# Autodesk Inventor assembly: 27t track drive sprocket
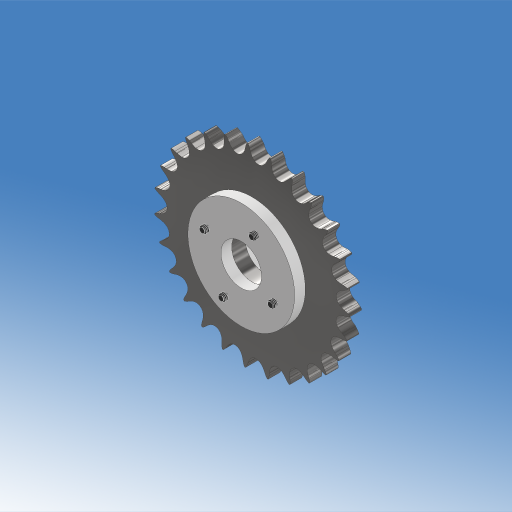
[picture p0: Inventor's stored thumbnail of the model, 512x512]
Saved by Autodesk Inventor 2024 (Build 280153000, 153)
## iProperties
Created: 2023-01-21
Part Number: 27t track drive sprocket
Document SubType Name: Assembly
Designer: AdminForWorker
Title: 27t track drive sprocket v25
Author: AdminForWorker
## Documents named in this file (5)
- C:\Users\seene\OneDrive\SBRT\Robocup Rescue\Drive\v1\TANK flipper\27t track drive sprocket v25.iam
- C:\Users\seene\OneDrive\SBRT\Robocup Rescue\Drive\v1\TANK flipper\91259A166_Alloy Steel Shoulder Screw v2.ipt
- C:\Users\seene\OneDrive\SBRT\Robocup Rescue\Drive\v1\TANK flipper\sprocket.ipt
- C:\Users\seene\OneDrive\SBRT\Robocup Rescue\Drive\v1\flipper dxf\drive sprocket flange.ipt
- C:\Users\seene\OneDrive\SBRT\Robocup Rescue\Drive\v1\flipper dxf\drive sprocket flange socket.ipt
## Components (7 placed, 4 different names)
1. 91259A166_Alloy Steel Shoulder Screw v2:5 — Rigid:4
2. 91259A166_Alloy Steel Shoulder Screw v2:6 — Rigid:3
3. 91259A166_Alloy Steel Shoulder Screw v2:7 — Rigid:2
4. 91259A166_Alloy Steel Shoulder Screw v2:8 — Rigid:1
5. sprocket:1 — Mate:1, Mate:2, Mate:3, Mate:4, Rigid:1, Rigid:2, Rigid:3, Rigid:4
6. drive sprocket flange:1 — Mate:3, Mate:4
7. drive sprocket flange socket:1 — Mate:1, Mate:2
## Relationships (8: Mate 4, WeldJoint 4)
- Mate:1: sprocket:1 ↔ drive sprocket flange socket:1
- Mate:2: sprocket:1 ↔ drive sprocket flange socket:1
- Mate:3: sprocket:1 ↔ drive sprocket flange:1
- Mate:4: sprocket:1 ↔ drive sprocket flange:1
- Rigid:1 [WeldJoint]: 91259A166_Alloy Steel Shoulder Screw v2:8 ↔ sprocket:1
- Rigid:2 [WeldJoint]: 91259A166_Alloy Steel Shoulder Screw v2:7 ↔ sprocket:1
- Rigid:3 [WeldJoint]: 91259A166_Alloy Steel Shoulder Screw v2:6 ↔ sprocket:1
- Rigid:4 [WeldJoint]: 91259A166_Alloy Steel Shoulder Screw v2:5 ↔ sprocket:1
